# Autodesk Inventor assembly: HbIndexFinger_flex01
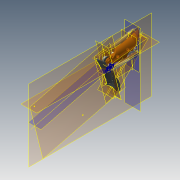
[picture p0: Inventor's stored thumbnail of the model, 180x180]
Saved by Autodesk Inventor 2015 SP1 (Build 190203100, 203)
## iProperties
Created: 2015-02-13
Part Number: HbIndexFinger_flex01
Document SubType Name: Assembly
Designer: Yamaura
Author: Yamaura
## Documents named in this file (11)
- C:\Users\Yamaura\Google ドライブ\exiii\3D\150405HackBerry\00_Latest\HbIndexFinger_flex01.iam
- C:\Users\Yamaura\Google ドライブ\exiii\3D\150405HackBerry\00_Latest\HbIndexMiddle-DistalPhalanx01.ipt
- C:\Users\Yamaura\Google ドライブ\exiii\3D\150405HackBerry\00_Latest\HbIndexInputLink01.ipt
- C:\Users\Yamaura\Google ドライブ\exiii\3D\150405HackBerry\00_Latest\HbIndexCouplerLink01.ipt
- C:\Users\Yamaura\Google ドライブ\exiii\3D\150405HackBerry\00_Latest\HbIndexCouplerLinkCover01.ipt
- C:\Users\Yamaura\Google ドライブ\exiii\3D\150405HackBerry\00_Latest\TOS 0.5-6-270-5.ipt
- C:\Users\Yamaura\Google ドライブ\exiii\3D\150405HackBerry\00_Latest\HbIndexMiddle-DistalPhalanxCover01.ipt
- C:\Users\Yamaura\Google ドライブ\exiii\3D\150405HackBerry\00_Latest\HbIndexPosture_flex01.ipt
- C:\Users\Yamaura\Google ドライブ\exiii\3D\150405HackBerry\00_Latest\HbReleaseLever01.ipt
- C:\Users\Yamaura\Google ドライブ\exiii\3D\150405HackBerry\00_Latest\HbIndexProximalPhalanx03.ipt
- C:\Users\Yamaura\Google ドライブ\exiii\3D\150405HackBerry\00_Latest\HbIndexProximalPhalanxCover02.ipt
## Components (11 placed, 10 different names)
1. HbIndexMiddle-DistalPhalanx01:1 — メイト:14, メイト:40, メイト:41
2. HbIndexPosture_flex01:1 — フラッシュ:2, フラッシュ:3, フラッシュ:4, メイト:14, メイト:15, メイト:35, メイト:36, メイト:29, メイト:38, メイト:39, メイト:40, メイト:45
3. HbIndexInputLink01:1 — メイト:7, フラッシュ:9, メイト:15, メイト:27, メイト:28
4. HbIndexCouplerLink01:1 — メイト:22, メイト:27, メイト:36
5. HbIndexCouplerLinkCover01:1 — フラッシュ:13, メイト:28, メイト:29
6. HbIndexProximalPhalanxCover02:1
7. TOS 0.5-6-270-5:1 — フラッシュ:15, メイト:35, フラッシュ:16, メイト:37
8. TOS 0.5-6-270-5:2 — フラッシュ:16, メイト:37
9. HbIndexMiddle-DistalPhalanxCover01:1 — メイト:38, フラッシュ:17, メイト:39
10. HbReleaseLever01:1 — フラッシュ:18, レバー角度
11. HbIndexProximalPhalanx03:1 — メイト:45
## Relationships (27: Mate 16, Flush 10, Angle 1)
- フラッシュ:2 [Flush]: HbIndexPosture_flex01:1
- フラッシュ:3 [Flush]: HbIndexPosture_flex01:1
- フラッシュ:4 [Flush]: HbIndexPosture_flex01:1
- メイト:7 [Mate]: HbIndexInputLink01:1
- フラッシュ:9 [Flush] (1.5 mm): HbIndexInputLink01:1
- メイト:14 [Mate]: HbIndexMiddle-DistalPhalanx01:1 ↔ HbIndexPosture_flex01:1
- メイト:15 [Mate]: HbIndexPosture_flex01:1 ↔ HbIndexInputLink01:1
- メイト:22 [Mate] (-5.55 mm): HbIndexCouplerLink01:1
- フラッシュ:13 [Flush] (-5.55 mm): HbIndexCouplerLinkCover01:1
- メイト:27 [Mate]: HbIndexInputLink01:1 ↔ HbIndexCouplerLink01:1
- メイト:28 [Mate]: HbIndexInputLink01:1 ↔ HbIndexCouplerLinkCover01:1
- メイト:29 [Mate]: HbIndexPosture_flex01:1 ↔ HbIndexCouplerLinkCover01:1
- [Flush] (5.55 mm): HbIndexProximalPhalanxCover02:1
- フラッシュ:15 [Flush] (-1.75 mm): TOS 0.5-6-270-5:1
- メイト:35 [Mate]: HbIndexPosture_flex01:1 ↔ TOS 0.5-6-270-5:1
- メイト:36 [Mate]: HbIndexPosture_flex01:1 ↔ HbIndexCouplerLink01:1
- フラッシュ:16 [Flush]: TOS 0.5-6-270-5:1 ↔ TOS 0.5-6-270-5:2
- メイト:37 [Mate]: TOS 0.5-6-270-5:1 ↔ TOS 0.5-6-270-5:2
- メイト:38 [Mate]: HbIndexPosture_flex01:1 ↔ HbIndexMiddle-DistalPhalanxCover01:1
- フラッシュ:17 [Flush] (3.45 mm): HbIndexMiddle-DistalPhalanxCover01:1
- メイト:39 [Mate]: HbIndexPosture_flex01:1 ↔ HbIndexMiddle-DistalPhalanxCover01:1
- メイト:40 [Mate]: HbIndexMiddle-DistalPhalanx01:1 ↔ HbIndexPosture_flex01:1
- メイト:41 [Mate] (-3.55 mm): HbIndexMiddle-DistalPhalanx01:1
- [Mate]: HbIndexProximalPhalanxCover02:1 ↔ HbIndexMiddle-DistalPhalanxCover01:1
- フラッシュ:18 [Flush]: HbReleaseLever01:1
- レバー角度 [Angle] (-5 deg): HbReleaseLever01:1
- メイト:45 [Mate]: HbIndexPosture_flex01:1 ↔ HbIndexProximalPhalanx03:1
